# Autodesk Inventor assembly: Head
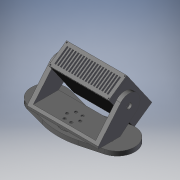
[picture p0: Inventor's stored thumbnail of the model, 180x180]
Saved by Autodesk Inventor 2017 SP1 (Build 210196100, 196)
## iProperties
Created: 2017-06-08
Part Number: Head
Document SubType Name: Assembly
Designer: zallen
Author: zallen
## Documents named in this file (9)
- C:\Users\Zach\Documents\GitHub\tr1\src\Head\Head.iam
- C:\Users\Zach\Documents\GitHub\tr1\src\Head\HA004.ipt
- C:\Users\Zach\Documents\GitHub\tr1\src\Head\HA006.ipt
- C:\Users\Zach\Documents\GitHub\tr1\lib\Xbox One Kinect\AS1.iam
- C:\Users\Zach\Documents\GitHub\tr1\src\Head\HA007.ipt
- C:\Users\Zach\Documents\GitHub\tr1\lib\DC Motor with Encoder\Motor.ipt
- C:\Users\Zach\Documents\GitHub\tr1\lib\4mm mounting hub.ipt
- C:\Users\Zach\Documents\GitHub\tr1\src\Head\HA009.ipt
- C:\Users\Zach\Documents\GitHub\tr1\src\Head\HA012.ipt
## Components (11 placed, 8 different names)
1. HA004:1 — Mate:49, Mate:50, Mate:61, Mate:73, Mate:74, Mate:78, Mate:79, Mate:80, Mate:82, Mate:93, Mate:94, Mate:95, Angle:1
2. HA006:1 — Mate:87, Mate:88, Mate:89
3. Kinect:1 [sub-assembly] — Mate:68, Mate:81, Mate:83
4. HA007:1 — Mate:84, Flush:1, Mate:85, Mate:86, Angle:1, Mate:96
5. Motor:1 — Mate:48, Mate:49, Mate:90
6. 4mm mounting hub:1 — Mate:48, Mate:50
7. HA009:1 — Mate:68, Mate:78, Mate:79, Mate:80, Mate:81, Mate:83, Mate:87, Mate:88, Mate:89, Mate:90, Mate:91, Mate:92, Angle:2
8. Motor:2 — Mate:91, Mate:92
9. 4mm mounting hub:2 — Mate:61, Mate:93, Mate:94
10. HA012:1 — Mate:73, Mate:74, Mate:75, Mate:76, Mate:77, Mate:82, Mate:84, Flush:1, Mate:95
11. 4mm mounting hub:3 — Mate:75, Mate:76, Mate:77
## Relationships (32: Mate 29, Angle 2, Flush 1)
- Mate:48: Motor:1 ↔ 4mm mounting hub:1
- Mate:49: HA004:1 ↔ Motor:1
- Mate:50: HA004:1 ↔ 4mm mounting hub:1
- Mate:61: HA004:1 ↔ 4mm mounting hub:2
- Mate:68: Kinect:1 ↔ HA009:1
- Mate:73: HA004:1 ↔ HA012:1
- Mate:74: HA004:1 ↔ HA012:1
- Mate:75: HA012:1 ↔ 4mm mounting hub:3
- Mate:76: HA012:1 ↔ 4mm mounting hub:3
- Mate:77: HA012:1 ↔ 4mm mounting hub:3
- Mate:78: HA004:1 ↔ HA009:1
- Mate:79 (5 mm): HA004:1 ↔ HA009:1
- Mate:80 (5 mm): HA004:1 ↔ HA009:1
- Mate:81: Kinect:1 ↔ HA009:1
- Mate:82: HA004:1 ↔ HA012:1
- Mate:83: Kinect:1 ↔ HA009:1
- Mate:84: HA007:1 ↔ HA012:1
- Flush:1: HA007:1 ↔ HA012:1
- Mate:85: HA007:1
- Mate:86: HA007:1
- Mate:87: HA006:1 ↔ HA009:1
- Mate:88: HA006:1 ↔ HA009:1
- Mate:89: HA006:1 ↔ HA009:1
- Mate:90: Motor:1 ↔ HA009:1
- Mate:91: HA009:1 ↔ Motor:2
- Mate:92: HA009:1 ↔ Motor:2
- Mate:93: HA004:1 ↔ 4mm mounting hub:2
- Mate:94: HA004:1 ↔ 4mm mounting hub:2
- Mate:95: HA004:1 ↔ HA012:1
- Angle:1 (180 deg): HA004:1 ↔ HA007:1
- Mate:96: HA007:1
- Angle:2 (15 deg): HA009:1
